# Autodesk Inventor assembly: BarcoFinal
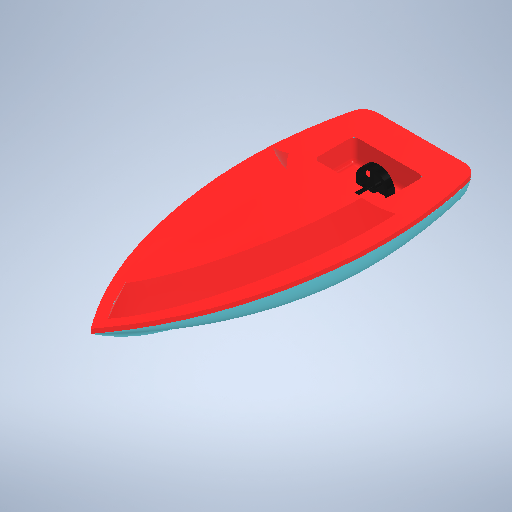
[picture p0: Inventor's stored thumbnail of the model, 512x512]
Saved by Autodesk Inventor 2025.1 (Build 291241000, 241)
## iProperties
Created: 2025-02-27
Part Number: BarcoFinal
Document SubType Name: Assembly
Designer: yovan
Author: yovan
## Documents named in this file (5)
- C:\Users\yovan\Desktop\APM\ausol-apm.github.io\project\Design and simulation\Inventor\Modelado juguetes\Barco\BarcoFinal.iam
- C:\Users\yovan\Desktop\APM\ausol-apm.github.io\project\Design and simulation\Inventor\Modelado juguetes\Barco\Inferior.ipt
- C:\Users\yovan\Desktop\APM\ausol-apm.github.io\project\Design and simulation\Inventor\Modelado juguetes\Barco\Piezabarcosuperior.ipt
- C:\Users\yovan\Desktop\APM\ausol-apm.github.io\project\Design and simulation\Inventor\Modelado juguetes\Barco\PiezaTimon.ipt
- C:\Users\yovan\Desktop\APM\ausol-apm.github.io\project\Design and simulation\Inventor\Modelado juguetes\Barco\Timon.ipt
## Components (4 placed, 4 different names)
1. Inferior:1 — Mate:4, Mate:5, Mate:6
2. Piezabarcosuperior:1 — Mate:1, Mate:2, Mate:3, Mate:4, Mate:5, Mate:6
3. PiezaTimon:1 — Insert:1
4. Timon:1 — Insert:1, Mate:1, Mate:2, Mate:3
## Relationships (7: Mate 6, Insert 1)
- Insert:1: PiezaTimon:1 ↔ Timon:1
- Mate:1: Piezabarcosuperior:1 ↔ Timon:1
- Mate:2: Piezabarcosuperior:1 ↔ Timon:1
- Mate:3: Piezabarcosuperior:1 ↔ Timon:1
- Mate:4: Inferior:1 ↔ Piezabarcosuperior:1
- Mate:5: Inferior:1 ↔ Piezabarcosuperior:1
- Mate:6: Inferior:1 ↔ Piezabarcosuperior:1
